# Autodesk Inventor assembly: CryptoWallet
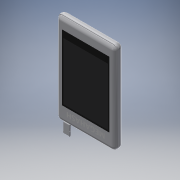
[picture p0: Inventor's stored thumbnail of the model, 180x180]
Saved by Autodesk Inventor 2017 (Build 210142000, 142)
## iProperties
Created: 2018-07-06
Part Number: CryptoWallet
Document SubType Name: Assembly
Designer: intelsath
Author: intelsath
## Documents named in this file (22)
- C:\Users\intelsath\Documents\Inventor\Cryptowallet\CryptoWallet.iam
- C:\Users\intelsath\Documents\Inventor\Cryptowallet\PCB.ipt
- C:\Users\intelsath\Documents\Inventor\Cryptowallet\LCD-Connector.ipt
- C:\Users\intelsath\Documents\Inventor\Cryptowallet\micro_usb_connector.iam
- C:\Users\intelsath\Documents\Inventor\Cryptowallet\MicroSD-holder.ipt
- C:\Users\intelsath\Documents\Inventor\Cryptowallet\Pogo-pin.ipt
- C:\Users\intelsath\Documents\Inventor\Cryptowallet\Push-button.ipt
- C:\Users\intelsath\Documents\Inventor\Cryptowallet\SiP.ipt
- C:\Users\intelsath\Documents\Inventor\Cryptowallet\QFN32.ipt
- C:\Users\intelsath\Documents\Inventor\Cryptowallet\SM02B-SRSS-TB.ipt
- C:\Users\intelsath\Documents\Inventor\Cryptowallet\Battery.ipt
- C:\Users\intelsath\Documents\Inventor\Cryptowallet\SHR-02V-S-B.ipt
- C:\Users\intelsath\Documents\Inventor\Cryptowallet\Antenna.ipt
- C:\Users\intelsath\Documents\Inventor\Cryptowallet\QFN24(4X4).ipt
- C:\Users\intelsath\Documents\Inventor\Cryptowallet\QFN-24 3x3 0.4mm.ipt
- C:\Users\intelsath\Documents\Inventor\Cryptowallet\Crystal 3225.ipt
- C:\Users\intelsath\Documents\Inventor\Cryptowallet\0603 LED v7.ipt
- C:\Users\intelsath\Documents\Inventor\Cryptowallet\Casing (Back).ipt
- C:\Users\intelsath\Documents\Inventor\Cryptowallet\Casing (Front).ipt
- C:\Users\intelsath\Documents\Inventor\Cryptowallet\LCD.iam
- C:\Users\intelsath\Documents\Inventor\Cryptowallet\Button Cap.ipt
- C:\Users\intelsath\Documents\Inventor\Cryptowallet\LED Pipe.ipt
## Components (24 placed, 21 different names)
1. PCB:1 — Mate:1, Flush:1, Flush:2, Mate:2, Mate:44, Mate:3, Mate:4, Mate:5, Flush:5, Flush:6, Flush:7, Mate:7, Mate:8, Flush:9, Flush:10, Tangent:1, Tangent:2, Flush:11, Flush:12, Mate:9, Mate:10, Flush:18, Flush:19, Flush:20, Flush:21, Mate:11, Flush:22, Flush:23, Mate:13, Mate:15, Mate:16, Mate:20, Flush:31, Flush:32, Mate:21, Mate:22, Flush:33, Flush:34, Flush:35, Flush:36, Mate:23, Flush:37, Flush:38, Mate:24, Flush:40, Mate:35, Mate:36, Mate:45, Flush:43, Flush:44
2. LCD-Connector:1 — Mate:1, Flush:1, Flush:2
3. micro_usb_connector:1 [sub-assembly] — Mate:2, Mate:44, Mate:45
4. MicroSD-holder:1 — Mate:3, Flush:5, Flush:6
5. Pogo-pin:1 — Mate:4, Flush:7, Mate:6, Flush:8
6. Pogo-pin:2 — Mate:5, Mate:6, Mate:7, Flush:8
7. Push-button:1 — Mate:8, Flush:9, Flush:10, Mate:43
8. SiP:1 — Tangent:1, Tangent:2, Flush:11, Flush:12
9. QFN32:1 — Mate:10, Flush:20, Flush:21
10. QFN32:2 — Mate:9, Flush:18, Flush:19
11. SM02B-SRSS-TB:1 — Mate:11, Flush:22, Flush:23, Mate:17, Mate:18, Mate:19
12. LCD:1 [sub-assembly] — Mate:13, Mate:14, Flush:45, Mate:50, Mate:51
13. Battery:1 — Mate:14, Mate:15, Mate:16, Flush:28, Mate:27, Mate:28, Mate:46
14. SHR-02V-S-B:1 — Mate:17, Mate:18, Mate:19, Mate:27, Mate:28
15. Antenna:1 — Flush:28, Flush:43, Flush:44
16. QFN24(4X4):1 — Mate:20, Flush:31, Flush:32
17. MPU-9250:1 — Mate:21, Flush:33, Flush:34
18. MPU-9250:2 — Mate:22, Flush:35, Flush:36
19. Crystal 3225:1 — Mate:23, Flush:37, Flush:38
20. 0603 LED v7:1 — Mate:24, Flush:40
21. Casing (Back):1 — Mate:35, Mate:36, Mate:46, Mate:48, Mate:49, Mate:52, Mate:53, Mate:54, Mate:55
22. Casing (Front):1 — Mate:49, Flush:45, Mate:50, Mate:51, Mate:52, Mate:53
23. Button Cap:1 — Mate:43
24. LED Pipe:1 — Mate:48, Mate:54, Mate:55
## Relationships (70: Mate 39, Flush 29, Tangent 2)
- Mate:1: PCB:1 ↔ LCD-Connector:1
- Flush:1 (2.35 mm): PCB:1 ↔ LCD-Connector:1
- Flush:2 (10.45 mm): PCB:1 ↔ LCD-Connector:1
- Mate:2: PCB:1 ↔ micro_usb_connector:1
- Mate:44 (-10.1 mm): PCB:1 ↔ micro_usb_connector:1
- Mate:3: PCB:1 ↔ MicroSD-holder:1
- Mate:4: PCB:1 ↔ Pogo-pin:1
- Mate:5: PCB:1 ↔ Pogo-pin:2
- Flush:5 (0.45 mm): PCB:1 ↔ MicroSD-holder:1
- Flush:6 (1.405 mm): PCB:1 ↔ MicroSD-holder:1
- Flush:7 (4.35 mm): PCB:1 ↔ Pogo-pin:1
- Mate:6 (3.2 mm): Pogo-pin:1 ↔ Pogo-pin:2
- Mate:7 (-32.85 mm): PCB:1 ↔ Pogo-pin:2
- Flush:8: Pogo-pin:1 ↔ Pogo-pin:2
- Mate:8: PCB:1 ↔ Push-button:1
- Flush:9 (0.25 mm): PCB:1 ↔ Push-button:1
- Flush:10 (24.75 mm): PCB:1 ↔ Push-button:1
- Tangent:1: PCB:1 ↔ SiP:1
- Tangent:2: PCB:1 ↔ SiP:1
- Flush:11 (0.4 mm): PCB:1 ↔ SiP:1
- Flush:12 (-10.3 mm): PCB:1 ↔ SiP:1
- Mate:9: PCB:1 ↔ QFN32:2
- Mate:10: PCB:1 ↔ QFN32:1
- Flush:18 (2.6 mm): PCB:1 ↔ QFN32:2
- Flush:19 (7.3 mm): PCB:1 ↔ QFN32:2
- Flush:20 (2.45 mm): PCB:1 ↔ QFN32:1
- Flush:21 (30.2 mm): PCB:1 ↔ QFN32:1
- Mate:11: PCB:1 ↔ SM02B-SRSS-TB:1
- Flush:22 (7.6 mm): PCB:1 ↔ SM02B-SRSS-TB:1
- Flush:23 (1.5 mm): PCB:1 ↔ SM02B-SRSS-TB:1
- Mate:13: PCB:1 ↔ LCD:1
- Mate:14: LCD:1 ↔ Battery:1
- Mate:15: PCB:1 ↔ Battery:1
- Mate:16: PCB:1 ↔ Battery:1
- Mate:17: SM02B-SRSS-TB:1 ↔ SHR-02V-S-B:1
- Mate:18: SM02B-SRSS-TB:1 ↔ SHR-02V-S-B:1
- Mate:19: SM02B-SRSS-TB:1 ↔ SHR-02V-S-B:1
- Flush:28: Battery:1 ↔ Antenna:1
- Mate:20: PCB:1 ↔ QFN24(4X4):1
- Flush:31 (2.7 mm): PCB:1 ↔ QFN24(4X4):1
- Flush:32 (3.5 mm): PCB:1 ↔ QFN24(4X4):1
- Mate:21: PCB:1 ↔ MPU-9250:1
- Mate:22: PCB:1 ↔ MPU-9250:2
- Flush:33 (10 mm): PCB:1 ↔ MPU-9250:1
- Flush:34 (2.7 mm): PCB:1 ↔ MPU-9250:1
- Flush:35 (17.1 mm): PCB:1 ↔ MPU-9250:2
- Flush:36 (6.5 mm): PCB:1 ↔ MPU-9250:2
- Mate:23: PCB:1 ↔ Crystal 3225:1
- Flush:37 (1.4 mm): PCB:1 ↔ Crystal 3225:1
- Flush:38 (2.75 mm): PCB:1 ↔ Crystal 3225:1
- Mate:24: PCB:1 ↔ 0603 LED v7:1
- Mate:27: Battery:1 ↔ SHR-02V-S-B:1
- Mate:28: Battery:1 ↔ SHR-02V-S-B:1
- Flush:40 (2.5 mm): PCB:1 ↔ 0603 LED v7:1
- Mate:35: PCB:1 ↔ Casing (Back):1
- Mate:36: PCB:1 ↔ Casing (Back):1
- Mate:43: Push-button:1 ↔ Button Cap:1
- Mate:45 (-4.4 mm): PCB:1 ↔ micro_usb_connector:1
- Flush:43 (4.9 mm): PCB:1 ↔ Antenna:1
- Flush:44 (32.05 mm): PCB:1 ↔ Antenna:1
- Mate:46: Battery:1 ↔ Casing (Back):1
- Mate:48: Casing (Back):1 ↔ LED Pipe:1
- Mate:49: Casing (Back):1 ↔ Casing (Front):1
- Flush:45: LCD:1 ↔ Casing (Front):1
- Mate:50: LCD:1 ↔ Casing (Front):1
- Mate:51: LCD:1 ↔ Casing (Front):1
- Mate:52: Casing (Back):1 ↔ Casing (Front):1
- Mate:53: Casing (Back):1 ↔ Casing (Front):1
- Mate:54: Casing (Back):1 ↔ LED Pipe:1
- Mate:55: Casing (Back):1 ↔ LED Pipe:1
